# Autodesk Inventor assembly: Assemlby_OpenOxygen
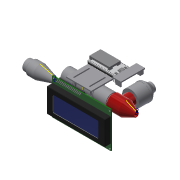
[picture p0: Inventor's stored thumbnail of the model, 180x180]
Saved by Autodesk Inventor 2019.4 (Build 234330000, 330)
## iProperties
Created: 2021-06-01
Part Number: Assemlby_OpenOxygen
Document SubType Name: Assembly
Designer: diederichbenedict
Author: diederichbenedict
## Documents named in this file (8)
- C:\Users\diederichbenedict\Dropbox\Dokumente\Promotion\PROJECTS\OXYGEN\INVENTOR\Assemlby_OpenOxygen.iam
- C:\Users\diederichbenedict\Dropbox\Dokumente\Promotion\PROJECTS\OXYGEN\INVENTOR\00_Sensirion_Flowsensor.ipt
- C:\Users\diederichbenedict\Dropbox\Dokumente\Promotion\PROJECTS\OXYGEN\INVENTOR\00_Arduino_LCD_I2Cstep.ipt
- C:\Users\diederichbenedict\Dropbox\Dokumente\Promotion\PROJECTS\OXYGEN\INVENTOR\00_ESP32.ipt
- C:\Users\diederichbenedict\Dropbox\Dokumente\Promotion\PROJECTS\OXYGEN\INVENTOR\00_Oxygen_Oxi.ipt
- C:\Users\diederichbenedict\Dropbox\Dokumente\Promotion\PROJECTS\OXYGEN\INVENTOR\00_LM286.ipt
- C:\Users\diederichbenedict\Dropbox\Dokumente\Promotion\PROJECTS\OXYGEN\INVENTOR\01_Connector_T.ipt
- C:\Users\diederichbenedict\Dropbox\Dokumente\Promotion\PROJECTS\OXYGEN\INVENTOR\02_Connector_S.ipt
## Components (7 placed, 7 different names)
1. 00_Sensirion_Flowsensor:1 — Flush:1, Angle:1, Flush:2, Flush:3, Flush:4, Insert:1
2. 00_Arduino_LCD_I2Cstep:1 — Flush:1, Angle:1, Flush:2
3. 00_ESP32:1 — Flush:3, Angle:3
4. 00_LM286:1 — Flush:4, Angle:3
5. 01_Connector_T:1 — Insert:1, Insert:2
6. 00_Oxygen_Oxi:1 — Insert:2
7. 02_Connector_S:1
## Relationships (8: Flush 4, Angle 2, Insert 2)
- Flush:1 (5 mm): 00_Sensirion_Flowsensor:1 ↔ 00_Arduino_LCD_I2Cstep:1
- Angle:1 (180 deg): 00_Sensirion_Flowsensor:1 ↔ 00_Arduino_LCD_I2Cstep:1
- Flush:2 (-10 mm): 00_Sensirion_Flowsensor:1 ↔ 00_Arduino_LCD_I2Cstep:1
- Flush:3: 00_Sensirion_Flowsensor:1 ↔ 00_ESP32:1
- Flush:4: 00_Sensirion_Flowsensor:1 ↔ 00_LM286:1
- Angle:3 (180 deg): 00_ESP32:1 ↔ 00_LM286:1
- Insert:1: 00_Sensirion_Flowsensor:1 ↔ 01_Connector_T:1
- Insert:2: 01_Connector_T:1 ↔ 00_Oxygen_Oxi:1
